# Autodesk Inventor assembly: surgical toolbox
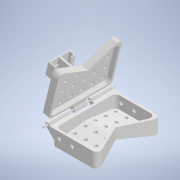
[picture p0: Inventor's stored thumbnail of the model, 180x180]
Saved by Autodesk Inventor 2020 (Build 240168000, 168)
## iProperties
Created: 2023-03-19
Part Number: surgical toolbox
Document SubType Name: Assembly
Designer: jcui7
Author: jcui7
## Documents named in this file (4)
- D:\InventorFiles\Get-a-Grip\surgical toolbox.iam
- D:\InventorFiles\Get-a-Grip\cylinder.ipt
- D:\InventorFiles\Get-a-Grip\general - Copy.ipt
- D:\InventorFiles\Get-a-Grip\general.ipt
## Components (3 placed, 3 different names)
1. cylinder:1 — Rotational:1
2. bottom — Rotational:1, Rotational:2
3. top — Rotational:2
## Relationships (2: RevoluteJoint 2)
- Rotational:1 [RevoluteJoint] (-2 mm): cylinder:1 ↔ bottom
- Rotational:2 [RevoluteJoint] (-2 mm): bottom ↔ top
